# Autodesk Inventor assembly: hand
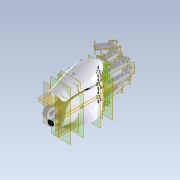
[picture p0: Inventor's stored thumbnail of the model, 180x180]
Saved by Autodesk Inventor 2020.2 (Build 242310000, 310)
## iProperties
Created: 2020-04-08
Part Number: hand
Document SubType Name: Assembly
Designer: Bardo91
thread_hole: 2.500 mm
Author: Bardo91
## Documents named in this file (25)
- D:\programming\elric\hardware\1. hand\elric20-01A.iam
- D:\programming\elric\hardware\1. hand\pinky_f1.ipt
- D:\programming\elric\hardware\1. hand\pinky_f2.ipt
- D:\programming\elric\hardware\1. hand\pinky_f3.ipt
- D:\programming\elric\hardware\1. hand\base_hand.ipt
- D:\programming\elric\hardware\1. hand\motor_dc_6v_30rpm.ipt
- D:\programming\elric\hardware\1. hand\finger_thread_lock.ipt
- D:\programming\elric\hardware\1. hand\finger_pulley.ipt
- D:\programming\elric\hardware\1. hand\ring_f2.ipt
- D:\programming\elric\hardware\1. hand\ring_f3.ipt
- D:\programming\elric\hardware\1. hand\ring_f1.ipt
- D:\programming\elric\hardware\1. hand\middle_f1.ipt
- D:\programming\elric\hardware\1. hand\middle_f2.ipt
- D:\programming\elric\hardware\1. hand\middle_f3.ipt
- D:\programming\elric\hardware\1. hand\index_f1.ipt
- D:\programming\elric\hardware\1. hand\index_f2.ipt
- D:\programming\elric\hardware\1. hand\index_f3.ipt
- D:\programming\elric\hardware\1. hand\thumb_f2.ipt
- D:\programming\elric\hardware\1. hand\thumb_f3.ipt
- D:\programming\elric\hardware\1. hand\thumb_f1.ipt
- D:\programming\elric\hardware\1. hand\cases\hand_case_1.ipt
- D:\programming\elric\hardware\1. hand\cases\hand_case_2.ipt
- D:\programming\elric\hardware\1. hand\cases\hand_case_3.ipt
- D:\programming\elric\hardware\1. hand\potentiometer_bourns_3382_12mm.ipt
- D:\programming\elric\hardware\1. hand\potentiometer_holder.ipt
## Components (39 placed, 24 different names)
1. base_hand:1 — Flush:9, Mate:12, Mate:32, Mate:33, Mate:36, Mate:37, Mate:40, Mate:41, Mate:78, Flush:18, Mate:79, Mate:80, Mate:81, Mate:83, Mate:84, Mate:85, Mate:87, Mate:88, Mate:89, Mate:92, Mate:93, Mate:94, Mate:95, Mate:96, Flush:19, Flush:20, Mate:98, Mate:99, Mate:100, Mate:102, Mate:103
2. potentiometer_bourns_3382_12mm:1 — Tangent:5, Mate:91
3. potentiometer_bourns_3382_12mm:2 — Tangent:4, Mate:90
4. potentiometer_bourns_3382_12mm:3 — Tangent:3, Mate:86
5. potentiometer_bourns_3382_12mm:4 — Tangent:6, Mate:101
6. potentiometer_bourns_3382_12mm:5 — Mate:77, Tangent:1
7. potentiometer_bourns_3382_12mm:6 — Tangent:2, Mate:82
8. potentiometer_holder:1 — Mate:79, Mate:80, Mate:81, Tangent:1
9. potentiometer_holder:2 — Tangent:3, Mate:86, Mate:87, Mate:88, Mate:89
10. potentiometer_holder:3 — Tangent:2, Mate:82, Mate:83, Mate:84, Mate:85
11. potentiometer_holder:4 — Tangent:4, Mate:90, Mate:98, Mate:99, Mate:100
12. potentiometer_holder:5 — Tangent:5, Mate:91, Mate:92, Mate:93, Mate:94
13. potentiometer_holder:6 — Tangent:6, Mate:101, Mate:102, Mate:103, Mate:104
14. hand_case_1:1
15. hand_case_2:1
16. hand_case_3:1
17. motor_dc_6v_30rpm:1 — Mate:77, Mate:78, Flush:18
18. finger_thread_lock:1 — Mate:25, Mate:26
19. pinky_f1:1 — Mate:1, Flush:1, Flush:9, Mate:12
20. pinky_f2:1 — Mate:1, Flush:1, Flush:2, Mate:2
21. pinky_f3:1 — Flush:2, Mate:2, Mate:25, Mate:26
22. motor_dc_6v_30rpm:2
23. ring_f2:1 — Mate:30, Mate:31, Flush:10, Flush:11
24. ring_f3:1 — Mate:30, Flush:10
25. ring_f1:1 — Mate:31, Flush:11, Mate:32, Mate:33
26. motor_dc_6v_30rpm:4
27. middle_f1:1 — Mate:35, Mate:36, Mate:37, Flush:12
28. middle_f2:1 — Mate:34, Mate:35, Flush:12, Flush:13
29. middle_f3:1 — Mate:34, Flush:13
30. motor_dc_6v_30rpm:3
31. index_f1:1 — Mate:39, Mate:40, Flush:15, Mate:41
32. index_f2:1 — Mate:38, Mate:39, Flush:14, Flush:15
33. index_f3:1 — Mate:38, Flush:14
34. motor_dc_6v_30rpm:5 — Mate:95, Flush:19, Mate:97
35. motor_dc_6v_30rpm:6 — Mate:67, Mate:68, Mate:96, Flush:20, Mate:104
36. finger_pulley:5 — Mate:67, Mate:68
37. thumb_f1:1 — Mate:61, Flush:17, Mate:97
38. thumb_f2:1 — Mate:60, Mate:61, Flush:16, Flush:17
39. thumb_f3:1 — Mate:60, Flush:16
## Relationships (69: Mate 49, Flush 14, Tangent 6)
- Mate:1: pinky_f1:1 ↔ pinky_f2:1
- Flush:1: pinky_f1:1 ↔ pinky_f2:1
- Flush:2: pinky_f2:1 ↔ pinky_f3:1
- Mate:2: pinky_f2:1 ↔ pinky_f3:1
- Flush:9: base_hand:1 ↔ pinky_f1:1
- Mate:12: base_hand:1 ↔ pinky_f1:1
- Mate:25: finger_thread_lock:1 ↔ pinky_f3:1
- Mate:26 (0.25 mm): finger_thread_lock:1 ↔ pinky_f3:1
- Mate:30: ring_f2:1 ↔ ring_f3:1
- Mate:31: ring_f2:1 ↔ ring_f1:1
- Flush:10: ring_f2:1 ↔ ring_f3:1
- Flush:11: ring_f2:1 ↔ ring_f1:1
- Mate:32: base_hand:1 ↔ ring_f1:1
- Mate:33: base_hand:1 ↔ ring_f1:1
- Mate:34: middle_f2:1 ↔ middle_f3:1
- Mate:35: middle_f1:1 ↔ middle_f2:1
- Mate:36: base_hand:1 ↔ middle_f1:1
- Mate:37: base_hand:1 ↔ middle_f1:1
- Flush:12: middle_f1:1 ↔ middle_f2:1
- Flush:13: middle_f2:1 ↔ middle_f3:1
- Mate:38: index_f2:1 ↔ index_f3:1
- Mate:39: index_f1:1 ↔ index_f2:1
- Mate:40: base_hand:1 ↔ index_f1:1
- Flush:14: index_f2:1 ↔ index_f3:1
- Flush:15: index_f1:1 ↔ index_f2:1
- Mate:41: base_hand:1 ↔ index_f1:1
- Mate:60: thumb_f2:1 ↔ thumb_f3:1
- Mate:61: thumb_f1:1 ↔ thumb_f2:1
- Flush:16: thumb_f2:1 ↔ thumb_f3:1
- Flush:17: thumb_f1:1 ↔ thumb_f2:1
- Mate:67: motor_dc_6v_30rpm:6 ↔ finger_pulley:5
- Mate:68 (2.5 mm): motor_dc_6v_30rpm:6 ↔ finger_pulley:5
- Mate:77: potentiometer_bourns_3382_12mm:5 ↔ motor_dc_6v_30rpm:1
- Mate:78: base_hand:1 ↔ motor_dc_6v_30rpm:1
- Flush:18: base_hand:1 ↔ motor_dc_6v_30rpm:1
- Mate:79: base_hand:1 ↔ potentiometer_holder:1
- Mate:80: base_hand:1 ↔ potentiometer_holder:1
- Mate:81: base_hand:1 ↔ potentiometer_holder:1
- Tangent:1: potentiometer_bourns_3382_12mm:5 ↔ potentiometer_holder:1
- Tangent:2: potentiometer_bourns_3382_12mm:6 ↔ potentiometer_holder:3
- Mate:82: potentiometer_bourns_3382_12mm:6 ↔ potentiometer_holder:3
- Mate:83: base_hand:1 ↔ potentiometer_holder:3
- Mate:84: base_hand:1 ↔ potentiometer_holder:3
- Mate:85: base_hand:1 ↔ potentiometer_holder:3
- Tangent:3: potentiometer_bourns_3382_12mm:3 ↔ potentiometer_holder:2
- Mate:86: potentiometer_bourns_3382_12mm:3 ↔ potentiometer_holder:2
- Mate:87: base_hand:1 ↔ potentiometer_holder:2
- Mate:88: base_hand:1 ↔ potentiometer_holder:2
- Mate:89: base_hand:1 ↔ potentiometer_holder:2
- Tangent:4: potentiometer_bourns_3382_12mm:2 ↔ potentiometer_holder:4
- Tangent:5: potentiometer_bourns_3382_12mm:1 ↔ potentiometer_holder:5
- Mate:90: potentiometer_bourns_3382_12mm:2 ↔ potentiometer_holder:4
- Mate:91: potentiometer_bourns_3382_12mm:1 ↔ potentiometer_holder:5
- Mate:92: base_hand:1 ↔ potentiometer_holder:5
- Mate:93: base_hand:1 ↔ potentiometer_holder:5
- Mate:94: base_hand:1 ↔ potentiometer_holder:5
- Mate:95: base_hand:1 ↔ motor_dc_6v_30rpm:5
- Mate:96: base_hand:1 ↔ motor_dc_6v_30rpm:6
- Flush:19: base_hand:1 ↔ motor_dc_6v_30rpm:5
- Flush:20 (5 mm): base_hand:1 ↔ motor_dc_6v_30rpm:6
- Mate:97: motor_dc_6v_30rpm:5 ↔ thumb_f1:1
- Mate:98: base_hand:1 ↔ potentiometer_holder:4
- Mate:99: base_hand:1 ↔ potentiometer_holder:4
- Mate:100: base_hand:1 ↔ potentiometer_holder:4
- Tangent:6: potentiometer_bourns_3382_12mm:4 ↔ potentiometer_holder:6
- Mate:101: potentiometer_bourns_3382_12mm:4 ↔ potentiometer_holder:6
- Mate:102: base_hand:1 ↔ potentiometer_holder:6
- Mate:103: base_hand:1 ↔ potentiometer_holder:6
- Mate:104: potentiometer_holder:6 ↔ motor_dc_6v_30rpm:6
## Named parameters: thread_hole = 2.5 mm
